# Autodesk Inventor assembly: Ensamblaje2
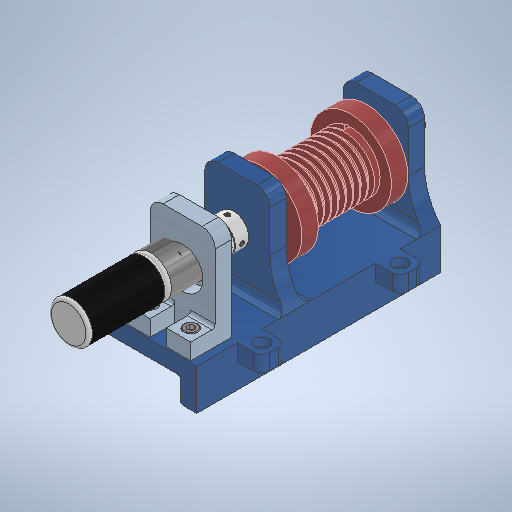
[picture p0: Inventor's stored thumbnail of the model, 512x512]
Saved by Autodesk Inventor 2026 (Build 300175050, 175E)
## iProperties
Created: 2025-06-30
Part Number: Ensamblaje2
Document SubType Name: Assembly
Designer: piero
Author: piero
## Documents named in this file (14)
- C:\Users\piero\OneDrive\Documentos\UTEC\Ciclo 2025-1\PFC_1\ModeloBase\CAD\Ensamblaje2.iam
- C:\Users\piero\OneDrive\Documentos\UTEC\Ciclo 2025-1\PFC_1\ModeloBase\CAD\soporte_inferior.ipt
- C:\Users\piero\OneDrive\Documentos\UTEC\Ciclo 2025-1\PFC_1\ModeloBase\CAD\acople_suave.ipt
- C:\Users\piero\OneDrive\Documentos\UTEC\Ciclo 2025-1\PFC_1\ModeloBase\CAD\Stepper Motor Nema 17_.ipt
- C:\Users\piero\OneDrive\Documentos\UTEC\Ciclo 2025-1\PFC_1\ModeloBase\CAD\perno_pasante.ipt
- C:\Users\piero\OneDrive\Documentos\UTEC\Ciclo 2025-1\PFC_1\ModeloBase\CAD\w_608-2rs1.iam
- C:\Users\piero\OneDrive\Documentos\UTEC\Ciclo 2025-1\PFC_1\ModeloBase\CAD\Brida1.ipt
- C:\Users\piero\OneDrive\Documentos\Inventor\Content Center Files\R2026\es-ES\AS 1421(4)\AS 1421 - M3 x 4 Punta plana.ipt
- C:\Users\piero\OneDrive\Documentos\UTEC\Ciclo 2025-1\PFC_1\ModeloBase\CAD\Motor.ipt
- C:\Users\piero\OneDrive\Documentos\UTEC\Ciclo 2025-1\PFC_1\ModeloBase\CAD\carrete.ipt
- C:\Users\piero\OneDrive\Documentos\UTEC\Ciclo 2025-1\PFC_1\ModeloBase\CAD\sujeción motor-acople.ipt
- C:\Users\piero\OneDrive\Documentos\Inventor\Content Center Files\R2026\es-ES\ANSI B18.6.3(05)\ANSI B18.6.3 - 4-40 UNC - 0.5(17).ipt
- C:\Users\piero\OneDrive\Documentos\Inventor\Content Center Files\R2026\es-ES\AS 1420\AS 1420 - 1973 - M5 x 20.ipt
- C:\Users\piero\OneDrive\Documentos\Inventor\Content Center Files\R2026\es-ES\AS 1112 (2)\AS 1112 - M5  Tipo 5.ipt
## Components (19 placed, 13 different names)
1. soporte_inferior:1 — Coincidencia:5, Coincidencia:8, De rotación:3, De rotación:4
2. acople_suave:2 — Coincidencia:6, Insertar:1, Insertar:2, Insertar:3, Coincidencia:16
3. Stepper Motor Nema 17_:2 — Coincidencia:8
4. perno_pasante:1 — Coincidencia:5, Coincidencia:6, Coincidencia:13, Coincidencia:14, Coincidencia:15, Coincidencia:19, Coincidencia:20
5. w_608-2rs1:1 [sub-assembly] — Coincidencia:13, De rotación:4
6. Brida1:1 — Coincidencia:14
7. Brida1:2 — Coincidencia:15
8. AS 1421 Punta plana - Métrico M3 x 4 Punta plana:1 — Insertar:1
9. AS 1421 Punta plana - Métrico M3 x 4 Punta plana:3 — Insertar:2
10. AS 1421 Punta plana - Métrico M3 x 4 Punta plana:4 — Insertar:3
11. AS 1421 Punta plana - Métrico M3 x 4 Punta plana:5 — Coincidencia:16
12. Motor:1 — Coincidencia:20
13. w_608-2rs1:3 [sub-assembly] — De rotación:3
14. carrete:1 — Coincidencia:19
15. sujeción motor-acople:1 — Insertar:5, Insertar:6, Nivelación:1, Coincidencia:21
16. Tornillo de fijación para maquinaria con hueco cruciforme - Tipo II - Pulgadas Nº 4 - 40 - 1/2:1 — Insertar:5
17. Tornillo de fijación para maquinaria con hueco cruciforme - Tipo II - Pulgadas Nº 4 - 40 - 1/2:2 — Insertar:6
18. AS 1420 - Métrico M5 x 20:1 — Coincidencia:21, Coincidencia:22
19. AS 1112 (2) - Métrico M5  Tipo 5:1 — Coincidencia:22
## Relationships (19: Mate 11, Insert 5, RevoluteJoint 2, Flush 1)
- Coincidencia:5 [Mate]: soporte_inferior:1 ↔ perno_pasante:1
- Coincidencia:6 [Mate]: acople_suave:2 ↔ perno_pasante:1
- Coincidencia:8 [Mate]: soporte_inferior:1 ↔ Stepper Motor Nema 17_:2
- Coincidencia:13 [Mate]: perno_pasante:1 ↔ w_608-2rs1:1
- Coincidencia:14 [Mate]: perno_pasante:1 ↔ Brida1:1
- Coincidencia:15 [Mate]: perno_pasante:1 ↔ Brida1:2
- Insertar:1: acople_suave:2 ↔ AS 1421 Punta plana - Métrico M3 x 4 Punta plana:1
- Insertar:2: acople_suave:2 ↔ AS 1421 Punta plana - Métrico M3 x 4 Punta plana:3
- Insertar:3: acople_suave:2 ↔ AS 1421 Punta plana - Métrico M3 x 4 Punta plana:4
- Coincidencia:16 [Mate]: acople_suave:2 ↔ AS 1421 Punta plana - Métrico M3 x 4 Punta plana:5
- De rotación:3 [RevoluteJoint]: soporte_inferior:1 ↔ w_608-2rs1:3
- Coincidencia:19 [Mate]: perno_pasante:1 ↔ carrete:1
- Coincidencia:20 [Mate]: perno_pasante:1 ↔ Motor:1
- Insertar:5: sujeción motor-acople:1 ↔ Tornillo de fijación para maquinaria con hueco cruciforme - Tipo II - Pulgadas Nº 4 - 40 - 1/2:1
- Insertar:6: sujeción motor-acople:1 ↔ Tornillo de fijación para maquinaria con hueco cruciforme - Tipo II - Pulgadas Nº 4 - 40 - 1/2:2
- Nivelación:1 [Flush] (-8 mm): sujeción motor-acople:1
- Coincidencia:21 [Mate]: sujeción motor-acople:1 ↔ AS 1420 - Métrico M5 x 20:1
- Coincidencia:22 [Mate]: AS 1420 - Métrico M5 x 20:1 ↔ AS 1112 (2) - Métrico M5  Tipo 5:1
- De rotación:4 [RevoluteJoint]: soporte_inferior:1 ↔ w_608-2rs1:1
